# Autodesk Inventor assembly: Forearm
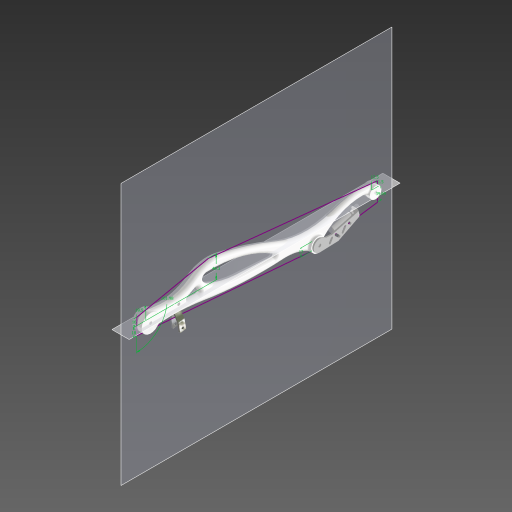
[picture p0: Inventor's stored thumbnail of the model, 512x512]
Saved by Autodesk Inventor 2023 (Build 270158000, 158)
## iProperties
Created: 2023-03-17
Part Number: Forearm
Document SubType Name: Assembly
Designer: valer
Author: valer
## Documents named in this file (5)
- C:\Users\Val\Desktop\drummingrobot\src\parts\export\Forearm.iam
- C:\Users\Val\Desktop\drummingrobot\src\parts\Forearm.ipt
- C:\Users\Val\Desktop\drummingrobot\src\parts\ForearmActuatorConnector.ipt
- C:\Users\Val\Desktop\drummingrobot\src\parts\SolenoidBracket.ipt
- C:\Users\Val\Desktop\drummingrobot\src\parts\external\ArmSolenoid.ipt
## Components (5 placed, 4 different names)
1. Forearm:1 — Mate:1, Mate:2, Mate:6, Mate:7, Mate:8, Mate:9, Mate:12, Mate:13, Mate:14
2. ForearmActuatorConnector:1 — Mate:6, Mate:7, Flush:1
3. SolenoidBracket:1 — Mate:1, Mate:2, Mate:10, Mate:11
4. ForearmActuatorConnector:2 — Mate:8, Mate:9, Flush:1
5. ArmSolenoid:1 — Mate:10, Mate:11
## Relationships (12: Mate 11, Flush 1)
- Mate:1: Forearm:1 ↔ SolenoidBracket:1
- Mate:2: Forearm:1 ↔ SolenoidBracket:1
- Mate:6: Forearm:1 ↔ ForearmActuatorConnector:1
- Mate:7: Forearm:1 ↔ ForearmActuatorConnector:1
- Mate:8: Forearm:1 ↔ ForearmActuatorConnector:2
- Mate:9: Forearm:1 ↔ ForearmActuatorConnector:2
- Flush:1: ForearmActuatorConnector:1 ↔ ForearmActuatorConnector:2
- Mate:10: SolenoidBracket:1 ↔ ArmSolenoid:1
- Mate:11: SolenoidBracket:1 ↔ ArmSolenoid:1
- Mate:12: Forearm:1
- Mate:13: Forearm:1
- Mate:14: Forearm:1
